# Autodesk Inventor assembly: union
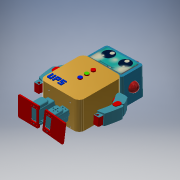
[picture p0: Inventor's stored thumbnail of the model, 180x180]
Saved by Autodesk Inventor 2017 (Build 210142000, 142)
## iProperties
Part Number: union
Material: Genérico
Document SubType Name: Assembly
Designer: Kevin
Author: Kevin
## Documents named in this file (10)
- C:\Users\Kevin\Desktop\tesisVero\brazoscuerpo\union.iam
- C:\Users\Kevin\Desktop\tesisVero\brazoscuerpo\CUERPO-VALIDO (1).ipt
- C:\Users\Kevin\Desktop\tesisVero\brazoscuerpo\brazocuadrado.ipt
- C:\Users\Kevin\Desktop\tesisVero\brazoscuerpo\cabeza2.ipt
- C:\Users\Kevin\Desktop\tesisVero\brazoscuerpo\antena.ipt
- C:\Users\Kevin\Desktop\tesis\MOSQUERA\DiseñoLucaz\EnsamblePierna.iam
- C:\Users\Kevin\Desktop\tesis\MOSQUERA\DiseñoLucaz\Base.ipt
- C:\Users\Kevin\Desktop\tesis\MOSQUERA\DiseñoLucaz\SERVO.iam
- C:\Users\Kevin\Desktop\tesis\MOSQUERA\DiseñoLucaz\Cielo.ipt
- C:\Users\Kevin\Desktop\tesis\MOSQUERA\DiseñoLucaz\BasePlacas.ipt
## Components (12 placed, 9 different names)
1. CUERPO-VALIDO (1):1 — De rotación:1, De rotación:2, De rotación:3, De rotación:4
2. brazocuadrado:1 — De rotación:2
3. brazocuadrado:2 — De rotación:1
4. cabeza2:1 — De rotación:3, Rígido:1
5. antena:1 — Rígido:1
6. EnsamblePierna:1 [sub-assembly] — De rotación:4
7. EnsamblePierna:4 [sub-assembly]
8. Base:2
9. SERVO:3 [sub-assembly]
10. SERVO:4 [sub-assembly]
11. Cielo:2
12. BasePlacas:1
## Relationships (5: RevoluteJoint 4, WeldJoint 1)
- De rotación:1 [RevoluteJoint] (8 mm): CUERPO-VALIDO (1):1 ↔ brazocuadrado:2
- De rotación:2 [RevoluteJoint] (7 mm): CUERPO-VALIDO (1):1 ↔ brazocuadrado:1
- De rotación:3 [RevoluteJoint] (6 mm): CUERPO-VALIDO (1):1 ↔ cabeza2:1
- Rígido:1 [WeldJoint]: cabeza2:1 ↔ antena:1
- De rotación:4 [RevoluteJoint] (1.5 mm): CUERPO-VALIDO (1):1 ↔ EnsamblePierna:1
